# Autodesk Inventor assembly: Pump System
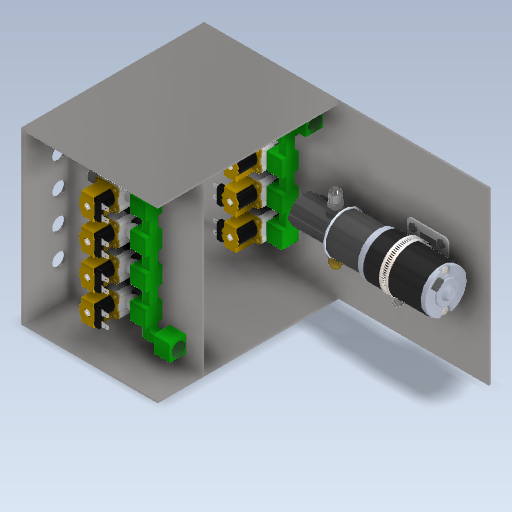
[picture p0: Inventor's stored thumbnail of the model, 512x512]
Saved by Autodesk Inventor 2020 (Build 240168000, 168)
## iProperties
Created: 2020-08-16
Part Number: Pump System
Document SubType Name: Assembly
Designer: Abbas
Author: Abbas
## Documents named in this file (5)
- C:\Users\LENOVO\Desktop\Graduation Project\Fish Farming Unit\Pump System\Pump System.iam
- C:\Users\LENOVO\Desktop\Graduation Project\Fish Farming Unit\Valves_Pump Holder\Valves_Pump Holder.ipt
- C:\Users\LENOVO\Desktop\Graduation Project\Fish Farming Unit\Water Loop Components\Pump_P-SERIES.iam
- C:\Users\LENOVO\Desktop\Graduation Project\Fish Farming Unit\Water Loop Components\valve_splitter_output.iam
- C:\Users\LENOVO\Desktop\Graduation Project\Fish Farming Unit\Water Loop Components\valve_splitter_input.iam
## Components (4 placed, 4 different names)
1. Valves_Pump Holder:2 — Insert:1, Mate:2, Mate:3, Insert:2, Insert:3
2. Pump_P-SERIES:1 [sub-assembly] — Insert:1
3. valve_splitter_output:1 [sub-assembly] — Mate:3, Insert:2
4. valve_splitter_input:1 [sub-assembly] — Mate:2, Insert:3
## Relationships (5: Insert 3, Mate 2)
- Insert:1: Valves_Pump Holder:2 ↔ Pump_P-SERIES:1
- Mate:2: Valves_Pump Holder:2 ↔ valve_splitter_input:1
- Mate:3: Valves_Pump Holder:2 ↔ valve_splitter_output:1
- Insert:2 (50 mm): Valves_Pump Holder:2 ↔ valve_splitter_output:1
- Insert:3 (50 mm): Valves_Pump Holder:2 ↔ valve_splitter_input:1
